# Autodesk Inventor assembly: 2ndAxis
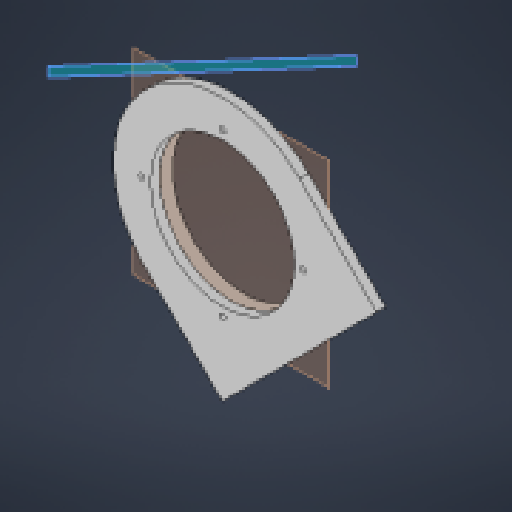
[picture p0: Inventor's stored thumbnail of the model, 512x512]
Saved by Autodesk Inventor 2024 (Build 280153000, 153)
## iProperties
Created: 2023-10-21
Part Number: 2ndAxis
Document SubType Name: Assembly
Designer: range
Author: range
## Documents named in this file (5)
- C:\Users\range\CodingProjects\C-AAM\CAD\V1\Parts\2ndAxis.iam
- C:\Users\range\CodingProjects\C-AAM\CAD\V1\Parts\TopSpacer.ipt
- C:\Users\range\CodingProjects\C-AAM\CAD\V1\Parts\AxisBoard.ipt
- C:\Users\range\CodingProjects\C-AAM\CAD\V1\Parts\SideBoard.ipt
- C:\Users\range\CodingProjects\C-AAM\CAD\V1\Parts\LazySusan.iam
## Components (4 placed, 4 different names)
1. TopSpacer:1 — Flush:1, Flush:2
2. AxisBoard:1 — Flush:1, Flush:2, Flush:3, Flush:4
3. SideBoard:1 — Flush:3, Flush:4, Flush:5
4. LazySusan:1 [sub-assembly] — Flush:5
## Relationships (5: Flush 5)
- Flush:1: TopSpacer:1 ↔ AxisBoard:1
- Flush:2: TopSpacer:1 ↔ AxisBoard:1
- Flush:3: AxisBoard:1 ↔ SideBoard:1
- Flush:4: AxisBoard:1 ↔ SideBoard:1
- Flush:5: SideBoard:1 ↔ LazySusan:1
